# Autodesk Inventor assembly: main
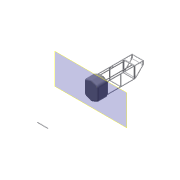
[picture p0: Inventor's stored thumbnail of the model, 180x180]
Saved by Autodesk Inventor 2014 SP1 (Build 180222100, 222)
## iProperties
Created: 2015-02-04
Part Number: main
Document SubType Name: Assembly
Designer: Simen
Author: Simen
## Documents named in this file (4)
- C:\Users\Simen\Documents\git\Eit\skjellet\main.iam
- C:\Users\Simen\Documents\git\Eit\skjellet\base.iam
- C:\Users\Simen\Documents\git\Eit\skjellet\skellett.iam
- C:\Users\Simen\Documents\git\Eit\skjellet\Head.iam
## Components (3 placed, 3 different names)
1. base:1 [sub-assembly] — Mate:5, Flush:16, Flush:17, Mate:7, Mate:8
2. skellett:1 [sub-assembly] — Mate:5, Flush:16, Flush:17, Mate:6, Flush:20, Flush:21
3. Head:1 [sub-assembly] — Mate:6, Flush:20, Flush:21
## Relationships (8: Mate 4, Flush 4)
- Mate:5: base:1 ↔ skellett:1
- Flush:16 (6 mm): base:1 ↔ skellett:1
- Flush:17 (92 mm): base:1 ↔ skellett:1
- Mate:6: skellett:1 ↔ Head:1
- Mate:7: base:1
- Mate:8: base:1
- Flush:20: skellett:1 ↔ Head:1
- Flush:21: skellett:1 ↔ Head:1
